# Autodesk Inventor assembly: horn_gear_2
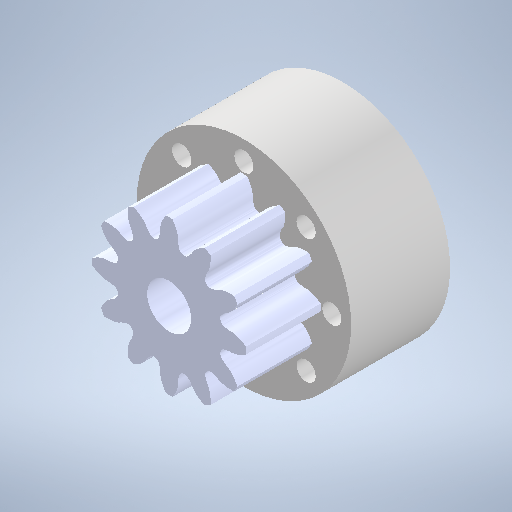
[picture p0: Inventor's stored thumbnail of the model, 512x512]
Saved by Autodesk Inventor 2025.2 (Build 292293000, 293)
## iProperties
Created: 2025-02-26
Part Number: horn_gear_2
Document SubType Name: Assembly
Designer: Admin
Author: Admin
## Documents named in this file (3)
- C:\Users\Admin\Desktop\Masters_Thesis_SDU\exoskeleton\horn_gear_2.iam
- C:\Users\Admin\Desktop\Masters_Thesis_SDU\exoskeleton\horn_3.ipt
- C:\Users\Admin\Desktop\Masters_Thesis_SDU\exoskeleton\gear_2.ipt
## Components (2 placed, 2 different names)
1. horn_3:1 — Mate:1, Mate:2
2. gear_2:1 — Mate:1, Mate:2
## Relationships (2: Mate 2)
- Mate:1: horn_3:1 ↔ gear_2:1
- Mate:2: horn_3:1 ↔ gear_2:1
